# Autodesk Inventor assembly: REC
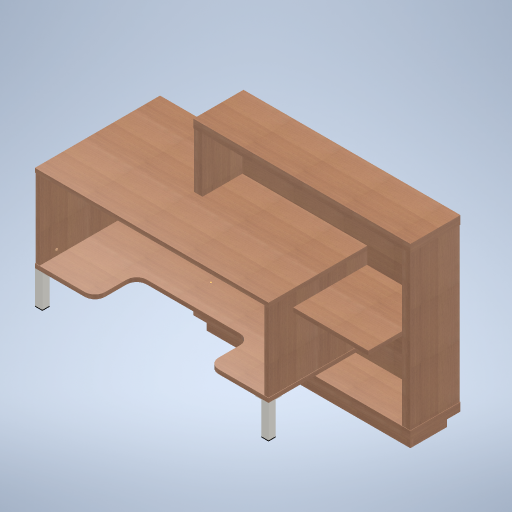
[picture p0: Inventor's stored thumbnail of the model, 512x512]
Saved by Autodesk Inventor 2024.3 (Build 283343000, 343)
## iProperties
Created: 2014-04-13
Part Number: REC
Document SubType Name: Assembly
Designer: SauliusD
Description: Reception
Material Code: Item.FillWorkpiece.Material.Code
Author: SauliusD
## Documents named in this file (28)
- C:\W4INV 2024 Design\PROJECTS\Samples\Simple Recepction\REC.iam
- C:\W4INV 2024 Design\PROJECTS\Samples\Simple Recepction\REC_00.ipt
- C:\W4INV 2024 Design\PROJECTS\Samples\Simple Recepction\REC_19.ipt
- C:\W4INV 2024 Design\PROJECTS\Samples\Simple Recepction\REC_18.ipt
- C:\W4INV 2024 Design\PROJECTS\Samples\Simple Recepction\REC_20.ipt
- C:\W4INV 2024 Design\PROJECTS\Samples\Simple Recepction\REC_17.ipt
- C:\W4INV 2024 Design\PROJECTS\Samples\Simple Recepction\REC_14.ipt
- C:\W4INV 2024 Design\PROJECTS\Samples\Simple Recepction\REC_13.ipt
- C:\W4INV 2024 Design\PROJECTS\Samples\Simple Recepction\REC_15.ipt
- C:\W4INV 2024 Design\PROJECTS\Samples\Simple Recepction\REC_11.ipt
- C:\W4INV 2024 Design\PROJECTS\Samples\Simple Recepction\REC_12.ipt
- C:\W4INV 2024 Design\PROJECTS\Samples\Simple Recepction\REC_10.ipt
- C:\W4INV 2024 Design\PROJECTS\Samples\Simple Recepction\REC_07.ipt
- C:\W4INV 2024 Design\PROJECTS\Samples\Simple Recepction\REC_06.ipt
- C:\W4INV 2024 Design\PROJECTS\Samples\Simple Recepction\REC_09.ipt
- C:\W4INV 2024 Design\PROJECTS\Samples\Simple Recepction\REC_08.ipt
- C:\W4INV 2024 Design\PROJECTS\Samples\Simple Recepction\REC_16.ipt
- C:\W4INV 2024 Design\_LIBRARY\Fixed joints\Confirmat\CONFIRMAT\Confirmat L70 & Cap D10 NB T40 PB T 40.ipt
- C:\W4INV 2024 Design\_LIBRARY\Fixed joints\Confirmat\CONFIRMAT\Confirmat L50 & Cap D10 NB T25 PB T 25.ipt
- C:\W4INV 2024 Design\_LIBRARY\Fixed joints\Minifix joint\MINIFIX D15 v2\Minifix D15 & Dowel L34 & Cap D15 PB T18 LH.ipt
- C:\W4INV 2024 Design\_LIBRARY\Fixed joints\Minifix joint\MINIFIX D15 v2\Minifix D15 & Dowel L34 & Cap D15 PB T18 RH.ipt
- C:\W4INV 2024 Design\PROJECTS\Samples\Simple Recepction\Minifixes pull Top Board-01.ipt
- C:\W4INV 2024 Design\PROJECTS\Samples\Simple Recepction\Minifixes pull Top Board-02.ipt
- C:\W4INV 2024 Design\PROJECTS\Samples\Simple Recepction\Minifixes pull Side Boards-04.ipt
- C:\W4INV 2024 Design\_LIBRARY\Supports and legs\Legs\RECTANGULAR LEG\Rectangular leg H200.ipt
- C:\W4INV 2024 Design\LIBRARY\Fixed joints\Confirmat\CONFIRMAT.ipt
- C:\W4INV 2024 Design\LIBRARY\Fixed joints\Minifix joint\MINIFIX D15 v2.ipt
- C:\W4INV 2024 Design\LIBRARY\Supports and legs\Legs\RECTANGULAR LEG.ipt
## Components (43 placed, 24 different names)
1. REC_00:1 — Flush:63, Flush:64, Flush:78, Flush:79, Mate:126, Mate:134
2. REC_19:1 — Flush:4, Flush:5, Flush:107, Flush:108
3. REC_18:1 — Flush:1, Flush:2, Flush:3, Flush:84, Flush:85, Mate:122, Mate:137, Bottom board plane:1, Bottom board plane:2, Angle Plane:2, Angle Plane:1, Bottom board plane:3, Angle Plane:3
4. REC_20:1 — Flush:65, Flush:66, Mate:125
5. REC_17:1 — Flush:111, Mate:135, Mate:136
6. REC_14:1 — Mate:128
7. REC_13:1 — Mate:99, Mate:131, Flush:110
8. REC_15:1 — Flush:6, Flush:7, Mate:2, Mate:4, Mate:83, Mate:85, Flush:109
9. REC_11:1 — Mate:109, Mate:111, Mate:113, Mate:115, Mate:117, Mate:119, Mate:132
10. REC_12:1
11. REC_10:1 — Mate:31, Mate:32, Mate:33, Mate:34
12. REC_07:1 — Mate:100, Mate:104, Mate:108, Flush:97, Mate:110, Mate:112, Flush:99, Mate:114, Mate:116, Flush:101, Mate:118
13. REC_06:1 — Mate:102, Mate:106, Flush:98, Flush:100, Flush:102
14. REC_09:1 — Flush:95, Flush:96
15. REC_08:1 — Flush:92, Flush:93, Flush:94
16. REC_16:1 — Flush:8, Mate:6, Mate:8, Flush:91
17. Confirmat L70 & Cap D10 NB T40 PB T 40:2 — Mate:1, Flush:63, Mate:2
18. Confirmat L70 & Cap D10 NB T40 PB T 40:3 — Mate:3, Flush:64, Mate:4
19. Confirmat L50 & Cap D10 NB T25 PB T 25:5 — Flush:65, Mate:6, Mate:65
20. Confirmat L50 & Cap D10 NB T25 PB T 25:6 — Mate:7, Flush:66, Mate:8
21. Confirmat L50 & Cap D10 NB T25 PB T 25:19 — Mate:31, Flush:78, Mate:32
22. Confirmat L50 & Cap D10 NB T25 PB T 25:20 — Mate:33, Flush:79, Mate:34
23. Confirmat L50 & Cap D10 NB T25 PB T 25:21 — Mate:82, Flush:84, Mate:83
24. Confirmat L50 & Cap D10 NB T25 PB T 25:22 — Mate:84, Flush:85, Mate:85
25. Minifix D15 & Dowel L34 & Cap D15 PB T18 RH:4 — Mate:98, Mate:99, Flush:91
26. Minifix D15 & Dowel L34 & Cap D15 PB T18 LH:5 — Flush:93, Mate:100, Mate:101
27. Minifix D15 & Dowel L34 & Cap D15 PB T18 RH:6 — Flush:94, Mate:102, Mate:103
28. Minifix D15 & Dowel L34 & Cap D15 PB T18 RH:7 — Flush:95, Mate:104, Mate:105
29. Minifix D15 & Dowel L34 & Cap D15 PB T18 LH:8 — Flush:96, Mate:106, Mate:107
30. Minifix D15 & Dowel L34 & Cap D15 PB T18 RH:10 — Mate:108, Flush:97, Mate:109
31. Minifix D15 & Dowel L34 & Cap D15 PB T18 LH:11 — Mate:110, Flush:98, Mate:111
32. Minifix D15 & Dowel L34 & Cap D15 PB T18 RH:12 — Mate:112, Flush:99, Mate:113
33. Minifix D15 & Dowel L34 & Cap D15 PB T18 RH:13 — Mate:114, Flush:100, Mate:115
34. Minifix D15 & Dowel L34 & Cap D15 PB T18 LH:14 — Mate:116, Flush:101, Mate:117
35. Minifix D15 & Dowel L34 & Cap D15 PB T18 RH:15 — Mate:118, Flush:102, Mate:119
36. Minifixes pull Top Board-01:1 — Mate:122, Flush:107, Mate:123, Mate:124, Mate:125
37. Minifixes pull Top Board-01:2 — Mate:126, Flush:108, Mate:127
38. Minifixes pull Top Board-02:1 — Mate:128, Flush:109, Mate:129, Mate:130, Mate:131
39. Minifixes pull Top Board-02:2 — Mate:132, Flush:110, Mate:133
40. Minifixes pull Side Boards-04:1 — Flush:111, Mate:134, Mate:135, Mate:136, Mate:137
41. Rectangular leg H200:1 — Y Axis Plane:1, Bottom board plane:1, X Axis Plane:1, Angle Plane:1
42. Rectangular leg H200:2 — Y Axis Plane:2, Bottom board plane:2, Angle Plane:2, X Axis Plane:2
43. Rectangular leg H200:3 — Bottom board plane:3, X Axis Plane:3, Y Axis Plane:3, Angle Plane:3
## Relationships (101: Mate 63, Flush 35, Angle 3)
- Flush:1 (-40 mm): REC_18:1
- Flush:2 (-40 mm): REC_18:1
- Flush:3 (-40 mm): REC_18:1
- Flush:4 (-100 mm): REC_19:1
- Flush:5 (-100 mm): REC_19:1
- Flush:6 (-100 mm): REC_15:1
- Flush:7 (-60 mm): REC_15:1
- Flush:8 (-80 mm): REC_16:1
- Flush:61 (-16 mm)
- Flush:62 (-16 mm)
- Mate:1: Confirmat L70 & Cap D10 NB T40 PB T 40:2
- Flush:63: REC_00:1 ↔ Confirmat L70 & Cap D10 NB T40 PB T 40:2
- Mate:2: REC_15:1 ↔ Confirmat L70 & Cap D10 NB T40 PB T 40:2
- Mate:3: Confirmat L70 & Cap D10 NB T40 PB T 40:3
- Flush:64: REC_00:1 ↔ Confirmat L70 & Cap D10 NB T40 PB T 40:3
- Mate:4: REC_15:1 ↔ Confirmat L70 & Cap D10 NB T40 PB T 40:3
- Flush:65: REC_20:1 ↔ Confirmat L50 & Cap D10 NB T25 PB T 25:5
- Mate:6 (-12.5 mm): REC_16:1 ↔ Confirmat L50 & Cap D10 NB T25 PB T 25:5
- Mate:7: Confirmat L50 & Cap D10 NB T25 PB T 25:6
- Flush:66: REC_20:1 ↔ Confirmat L50 & Cap D10 NB T25 PB T 25:6
- Mate:8 (-12.5 mm): REC_16:1 ↔ Confirmat L50 & Cap D10 NB T25 PB T 25:6
- Mate:31: REC_10:1 ↔ Confirmat L50 & Cap D10 NB T25 PB T 25:19
- Flush:78: REC_00:1 ↔ Confirmat L50 & Cap D10 NB T25 PB T 25:19
- Mate:32 (-12.5 mm): REC_10:1 ↔ Confirmat L50 & Cap D10 NB T25 PB T 25:19
- Mate:33: REC_10:1 ↔ Confirmat L50 & Cap D10 NB T25 PB T 25:20
- Flush:79: REC_00:1 ↔ Confirmat L50 & Cap D10 NB T25 PB T 25:20
- Mate:34 (-12.5 mm): REC_10:1 ↔ Confirmat L50 & Cap D10 NB T25 PB T 25:20
- Mate:65: Confirmat L50 & Cap D10 NB T25 PB T 25:5
- Mate:82: Confirmat L50 & Cap D10 NB T25 PB T 25:21
- Flush:84: REC_18:1 ↔ Confirmat L50 & Cap D10 NB T25 PB T 25:21
- Mate:83: REC_15:1 ↔ Confirmat L50 & Cap D10 NB T25 PB T 25:21
- Mate:84: Confirmat L50 & Cap D10 NB T25 PB T 25:22
- Flush:85: REC_18:1 ↔ Confirmat L50 & Cap D10 NB T25 PB T 25:22
- Mate:85: REC_15:1 ↔ Confirmat L50 & Cap D10 NB T25 PB T 25:22
- Mate:98: Minifix D15 & Dowel L34 & Cap D15 PB T18 RH:4
- Mate:99: REC_13:1 ↔ Minifix D15 & Dowel L34 & Cap D15 PB T18 RH:4
- Flush:91 (18 mm): REC_16:1 ↔ Minifix D15 & Dowel L34 & Cap D15 PB T18 RH:4
- Flush:92 (-20 mm): REC_08:1
- Flush:93 (18 mm): REC_08:1 ↔ Minifix D15 & Dowel L34 & Cap D15 PB T18 LH:5
- Mate:100: REC_07:1 ↔ Minifix D15 & Dowel L34 & Cap D15 PB T18 LH:5
- Mate:101: Minifix D15 & Dowel L34 & Cap D15 PB T18 LH:5
- Flush:94 (18 mm): REC_08:1 ↔ Minifix D15 & Dowel L34 & Cap D15 PB T18 RH:6
- Mate:102: REC_06:1 ↔ Minifix D15 & Dowel L34 & Cap D15 PB T18 RH:6
- Mate:103: Minifix D15 & Dowel L34 & Cap D15 PB T18 RH:6
- Flush:95 (18 mm): REC_09:1 ↔ Minifix D15 & Dowel L34 & Cap D15 PB T18 RH:7
- Mate:104: REC_07:1 ↔ Minifix D15 & Dowel L34 & Cap D15 PB T18 RH:7
- Mate:105: Minifix D15 & Dowel L34 & Cap D15 PB T18 RH:7
- Flush:96 (18 mm): REC_09:1 ↔ Minifix D15 & Dowel L34 & Cap D15 PB T18 LH:8
- Mate:106: REC_06:1 ↔ Minifix D15 & Dowel L34 & Cap D15 PB T18 LH:8
- Mate:107: Minifix D15 & Dowel L34 & Cap D15 PB T18 LH:8
- Mate:108: REC_07:1 ↔ Minifix D15 & Dowel L34 & Cap D15 PB T18 RH:10
- Flush:97 (18 mm): REC_07:1 ↔ Minifix D15 & Dowel L34 & Cap D15 PB T18 RH:10
- Mate:109: REC_11:1 ↔ Minifix D15 & Dowel L34 & Cap D15 PB T18 RH:10
- Mate:110: REC_07:1 ↔ Minifix D15 & Dowel L34 & Cap D15 PB T18 LH:11
- Flush:98 (18 mm): REC_06:1 ↔ Minifix D15 & Dowel L34 & Cap D15 PB T18 LH:11
- Mate:111: REC_11:1 ↔ Minifix D15 & Dowel L34 & Cap D15 PB T18 LH:11
- Mate:112: REC_07:1 ↔ Minifix D15 & Dowel L34 & Cap D15 PB T18 RH:12
- Flush:99 (18 mm): REC_07:1 ↔ Minifix D15 & Dowel L34 & Cap D15 PB T18 RH:12
- Mate:113: REC_11:1 ↔ Minifix D15 & Dowel L34 & Cap D15 PB T18 RH:12
- Mate:114: REC_07:1 ↔ Minifix D15 & Dowel L34 & Cap D15 PB T18 RH:13
- Flush:100 (18 mm): REC_06:1 ↔ Minifix D15 & Dowel L34 & Cap D15 PB T18 RH:13
- Mate:115: REC_11:1 ↔ Minifix D15 & Dowel L34 & Cap D15 PB T18 RH:13
- Mate:116: REC_07:1 ↔ Minifix D15 & Dowel L34 & Cap D15 PB T18 LH:14
- Flush:101 (18 mm): REC_07:1 ↔ Minifix D15 & Dowel L34 & Cap D15 PB T18 LH:14
- Mate:117: REC_11:1 ↔ Minifix D15 & Dowel L34 & Cap D15 PB T18 LH:14
- Mate:118: REC_07:1 ↔ Minifix D15 & Dowel L34 & Cap D15 PB T18 RH:15
- Flush:102 (18 mm): REC_06:1 ↔ Minifix D15 & Dowel L34 & Cap D15 PB T18 RH:15
- Mate:119: REC_11:1 ↔ Minifix D15 & Dowel L34 & Cap D15 PB T18 RH:15
- Mate:122: REC_18:1 ↔ Minifixes pull Top Board-01:1
- Flush:107: REC_19:1 ↔ Minifixes pull Top Board-01:1
- Mate:123: Minifixes pull Top Board-01:1
- Mate:124: Minifixes pull Top Board-01:1
- Mate:125: REC_20:1 ↔ Minifixes pull Top Board-01:1
- Mate:126: REC_00:1 ↔ Minifixes pull Top Board-01:2
- Flush:108: REC_19:1 ↔ Minifixes pull Top Board-01:2
- Mate:127: Minifixes pull Top Board-01:2
- Mate:128: REC_14:1 ↔ Minifixes pull Top Board-02:1
- Flush:109: REC_15:1 ↔ Minifixes pull Top Board-02:1
- Mate:129: Minifixes pull Top Board-02:1
- Mate:130: Minifixes pull Top Board-02:1
- Mate:131: REC_13:1 ↔ Minifixes pull Top Board-02:1
- Mate:132: REC_11:1 ↔ Minifixes pull Top Board-02:2
- Flush:110: REC_13:1 ↔ Minifixes pull Top Board-02:2
- Mate:133: Minifixes pull Top Board-02:2
- Flush:111: REC_17:1 ↔ Minifixes pull Side Boards-04:1
- Mate:134: REC_00:1 ↔ Minifixes pull Side Boards-04:1
- Mate:135: REC_17:1 ↔ Minifixes pull Side Boards-04:1
- Mate:136: REC_17:1 ↔ Minifixes pull Side Boards-04:1
- Mate:137: REC_18:1 ↔ Minifixes pull Side Boards-04:1
- Y Axis Plane:1 [Mate]: Rectangular leg H200:1
- Bottom board plane:1 [Mate]: REC_18:1 ↔ Rectangular leg H200:1
- Y Axis Plane:2 [Mate]: Rectangular leg H200:2
- Bottom board plane:2 [Mate]: REC_18:1 ↔ Rectangular leg H200:2
- Angle Plane:2 (0 deg): REC_18:1 ↔ Rectangular leg H200:2
- X Axis Plane:1 [Mate]: Rectangular leg H200:1
- Angle Plane:1 (0 deg): REC_18:1 ↔ Rectangular leg H200:1
- X Axis Plane:2 [Mate]: Rectangular leg H200:2
- Bottom board plane:3 [Mate]: REC_18:1 ↔ Rectangular leg H200:3
- X Axis Plane:3 [Mate]: Rectangular leg H200:3
- Y Axis Plane:3 [Mate]: Rectangular leg H200:3
- Angle Plane:3 (0 deg): REC_18:1 ↔ Rectangular leg H200:3
